# Autodesk Inventor assembly: Main
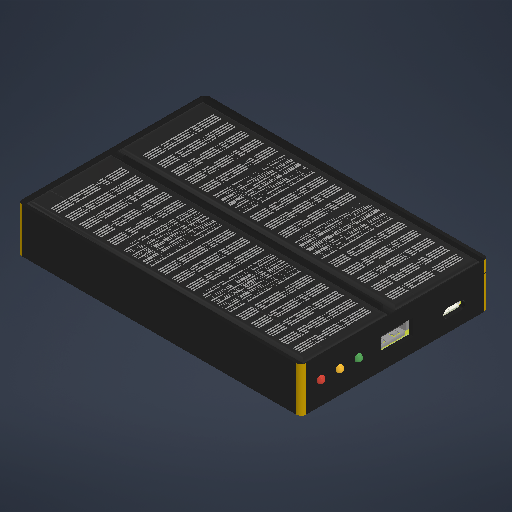
[picture p0: Inventor's stored thumbnail of the model, 512x512]
Saved by Autodesk Inventor 2027.1 (Build 311270010, 270A)
## iProperties
Created: 2026-09-18
Part Number: Main
Document SubType Name: Assembly
Designer: Rozkurwiator
Author: Rozkurwiator
## Documents named in this file (10)
- G:\Github\Solarbank\Hardware\Model\Main.iam
- G:\Github\Solarbank\Hardware\PCB\Power_bank_PCB\PCB\PCB\PCB.ipt
- G:\Github\Solarbank\Hardware\Model\Parts\Battery_prop.ipt
- G:\Github\Solarbank\Hardware\Model\Parts\Bottom.ipt
- G:\Github\Solarbank\Hardware\Model\Parts\led 3 mm amarillo\led 3 mm amarillo.ipt
- G:\Github\Solarbank\Hardware\Model\Parts\OscarML_Led 3mm Rojo v1\OscarML_Led 3mm Rojo v1.ipt
- G:\Github\Solarbank\Hardware\Model\Parts\OscarML_Led 3mm Verde\OscarML_Led 3mm Verde.ipt
- G:\Github\Solarbank\Hardware\Model\Parts\SolarPanel_30x65x3mm\SolarPanel_30x65x3mm.ipt
- G:\Github\Solarbank\Hardware\Model\Parts\Micro_Button_6x6\Micro_Button_6x6.ipt
- G:\Github\Solarbank\Hardware\Model\Parts\Top_part.ipt
## Components (20 placed, 9 different names)
1. PCB:1 — Obrotowe:1
2. Battery_prop:1 — Sztywne:1
3. Bottom:1 — Obrotowe:1, Sztywne:1, Obrotowe:2, Obrotowe:3, Obrotowe:4, Sztywne:2, Sztywne:3
4. led 3 mm amarillo:1 — Obrotowe:3
5. OscarML_Led 3mm Rojo v1:1 — Obrotowe:4
6. OscarML_Led 3mm Verde:1 — Obrotowe:2
7. Micro_Button_6x6:1 — Sztywne:2
8. Top_part:1 — Obrotowe:5, Sztywne:3
9. SolarPanel_30x65x3mm:1 — Obrotowe:5
10. SolarPanel_30x65x3mm:2
11. SolarPanel_30x65x3mm:3
12. SolarPanel_30x65x3mm:4
13. SolarPanel_30x65x3mm:5
14. SolarPanel_30x65x3mm:6
15. SolarPanel_30x65x3mm:7
16. SolarPanel_30x65x3mm:8
17. SolarPanel_30x65x3mm:9
18. SolarPanel_30x65x3mm:10
19. SolarPanel_30x65x3mm:11
20. SolarPanel_30x65x3mm:12
## Component patterns: (2 elements), (6 elements, first: SolarPanel_30x65x3mm:1), Szyk komponentów 1:2 (6 elements)
## Relationships (8: RevoluteJoint 5, WeldJoint 3)
- Obrotowe:1 [RevoluteJoint] (-1 mm): PCB:1 ↔ Bottom:1
- Sztywne:1 [WeldJoint] (5 mm): Battery_prop:1 ↔ Bottom:1
- Obrotowe:2 [RevoluteJoint]: Bottom:1 ↔ OscarML_Led 3mm Verde:1
- Obrotowe:3 [RevoluteJoint]: Bottom:1 ↔ led 3 mm amarillo:1
- Obrotowe:4 [RevoluteJoint]: Bottom:1 ↔ OscarML_Led 3mm Rojo v1:1
- Sztywne:2 [WeldJoint]: Bottom:1 ↔ Micro_Button_6x6:1
- Obrotowe:5 [RevoluteJoint]: Top_part:1 ↔ SolarPanel_30x65x3mm:1
- Sztywne:3 [WeldJoint] (-14 mm): Bottom:1 ↔ Top_part:1
